# Autodesk Inventor assembly: main climber
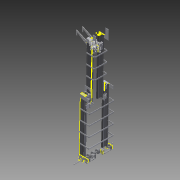
[picture p0: Inventor's stored thumbnail of the model, 180x180]
Saved by Autodesk Inventor 2013 (Build 170138000, 138)
## iProperties
Created: 2013-01-25
Part Number: main climber
Document SubType Name: Assembly
Designer: Arpan
Mass: 8247.06 g
Surface Area: 14203.7 cm^2
Volume: 3255.08 cm^3
Density: 2.53359 g/cm^3
Author: Arpan
## Documents named in this file (10)
- C:\Users\Arpan\Documents\GitHub\frc2013CAD\Cimber actual\main climber.iam
- C:\Users\Arpan\Documents\GitHub\frc2013CAD\Cimber actual\14 inch shaft.ipt
- C:\Users\Arpan\Documents\GitHub\frc2013CAD\Cimber actual\Inner rails.iam
- C:\Users\Arpan\Documents\GitHub\frc2013CAD\Cimber actual\outer rails.iam
- C:\Users\Arpan\Documents\GitHub\frc2013CAD\Cimber actual\small pulley assembly.iam
- C:\Users\Arpan\Documents\GitHub\frc2013CAD\Cimber actual\endstop 5.ipt
- C:\Users\Arpan\Documents\GitHub\frc2013CAD\Cimber actual\rough pulley.ipt
- C:\Users\Arpan\Documents\GitHub\frc2013CAD\Cimber actual\bottom pulley mount.ipt
- C:\Users\Arpan\Documents\GitHub\frc2013CAD\Cimber actual\Sideways pulley mount.iam
- C:\Users\Arpan\Documents\GitHub\frc2013CAD\Cimber actual\Sideways pulley mount 2.iam
## Components (14 placed, 9 different names)
1. Inner rails:1 [sub-assembly] — Mate:1, Angle:1, Flush:1, Mate:26, Mate:27, Flush:7
2. outer rails:1 [sub-assembly] — Mate:1, Mate:2, Angle:1, Flush:1, Flush:4, Mate:8, Mate:9, Mate:10, Mate:20, Mate:21, Mate:22, Mate:23, Mate:24, Mate:25, Mate:36, Flush:9, Mate:37, Flush:10, Flush:11, Mate:38, Mate:39
3. 14 inch shaft:1 — Mate:2, Flush:4, Mate:30, Mate:31, Mate:32
4. small pulley assembly:3 [sub-assembly] — Mate:8, Mate:9, Mate:10
5. small pulley assembly:8 [sub-assembly] — Mate:23, Mate:24, Mate:25
6. small pulley assembly:9 [sub-assembly] — Mate:20, Mate:21, Mate:22
7. endstop 5:2 — Mate:26, Mate:27
8. rough pulley:1 — Mate:31, Flush:8
9. rough pulley:2 — Mate:30, Mate:33
10. rough pulley:3 — Mate:32, Mate:35
11. bottom pulley mount:1 — Mate:37, Flush:10, Flush:11, Flush:12, Mate:40, Mate:41
12. bottom pulley mount:2 — Mate:36, Flush:9, Mate:38, Mate:39, Mate:45, Mate:46
13. Sideways pulley mount:1 [sub-assembly] — Flush:12, Mate:40, Mate:41, Flush:13
14. Sideways pulley mount 2:1 [sub-assembly] — Mate:45, Mate:46, Flush:13
## Relationships (36: Mate 26, Flush 9, Angle 1)
- Mate:1: Inner rails:1 ↔ outer rails:1
- Mate:2: outer rails:1 ↔ 14 inch shaft:1
- Angle:1 (180 deg): Inner rails:1 ↔ outer rails:1
- Flush:1 (508 mm): Inner rails:1 ↔ outer rails:1
- Flush:4 (-82.8929 mm): outer rails:1 ↔ 14 inch shaft:1
- Mate:8: outer rails:1 ↔ small pulley assembly:3
- Mate:9: outer rails:1 ↔ small pulley assembly:3
- Mate:10: outer rails:1 ↔ small pulley assembly:3
- Mate:20: outer rails:1 ↔ small pulley assembly:9
- Mate:21: outer rails:1 ↔ small pulley assembly:9
- Mate:22: outer rails:1 ↔ small pulley assembly:9
- Mate:23: outer rails:1 ↔ small pulley assembly:8
- Mate:24: outer rails:1 ↔ small pulley assembly:8
- Mate:25: outer rails:1 ↔ small pulley assembly:8
- Mate:26: Inner rails:1 ↔ endstop 5:2
- Mate:27: Inner rails:1 ↔ endstop 5:2
- Mate:30: 14 inch shaft:1 ↔ rough pulley:2
- Mate:31: 14 inch shaft:1 ↔ rough pulley:1
- Mate:32: 14 inch shaft:1 ↔ rough pulley:3
- Flush:7 (-6.35 mm): Inner rails:1
- Mate:33 (-10.3188 mm): rough pulley:2
- Mate:35 (-61.1188 mm): rough pulley:3
- Flush:8 (-61.1188 mm): rough pulley:1
- Mate:36: outer rails:1 ↔ bottom pulley mount:2
- Flush:9: outer rails:1 ↔ bottom pulley mount:2
- Mate:37: outer rails:1 ↔ bottom pulley mount:1
- Flush:10: outer rails:1 ↔ bottom pulley mount:1
- Flush:11 (12.192 mm): outer rails:1 ↔ bottom pulley mount:1
- Mate:38: outer rails:1 ↔ bottom pulley mount:2
- Mate:39: outer rails:1 ↔ bottom pulley mount:2
- Flush:12 (1.5875 mm): bottom pulley mount:1 ↔ Sideways pulley mount:1
- Mate:40: bottom pulley mount:1 ↔ Sideways pulley mount:1
- Mate:41: bottom pulley mount:1 ↔ Sideways pulley mount:1
- Mate:45: bottom pulley mount:2 ↔ Sideways pulley mount 2:1
- Mate:46: bottom pulley mount:2 ↔ Sideways pulley mount 2:1
- Flush:13: Sideways pulley mount:1 ↔ Sideways pulley mount 2:1
